# Autodesk Inventor assembly: terminal_MIR
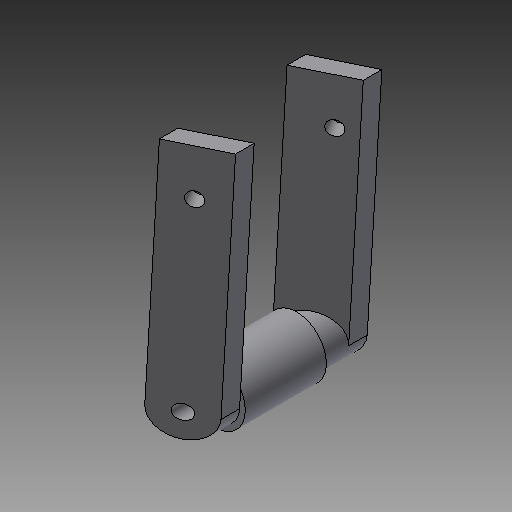
[picture p0: Inventor's stored thumbnail of the model, 512x512]
Saved by Autodesk Inventor 2018 (Build 220112000, 112)
## iProperties
Created: 2017-06-03
Part Number: terminal_MIR
Document SubType Name: Assembly
Designer: AYUSH SHUKLA
Author: AYUSH SHUKLA
## Documents named in this file (3)
- C:\Study\BTP2\Robomuse Inventor CAD\terminal_MIR.iam
- C:\Study\BTP2\Robomuse Inventor CAD\terminal_MIR.ipt
- C:\Study\BTP2\Robomuse Inventor CAD\terminal_mount_MIR.ipt
## Components (3 placed, 2 different names)
1. terminal_MIR:1 — Mate:1, Mate:4, Mate:2
2. terminal_mount_MIR:1 — Mate:1, Mate:3, Angle:1
3. terminal_mount_MIR:2 — Mate:4, Mate:3, Mate:2, Angle:1
## Relationships (5: Mate 4, Angle 1)
- Mate:1: terminal_MIR:1 ↔ terminal_mount_MIR:1
- Mate:4: terminal_MIR:1 ↔ terminal_mount_MIR:2
- Mate:3 (29.3294 mm): terminal_mount_MIR:1 ↔ terminal_mount_MIR:2
- Mate:2: terminal_MIR:1 ↔ terminal_mount_MIR:2
- Angle:1 (0 deg): terminal_mount_MIR:1 ↔ terminal_mount_MIR:2
